# Autodesk Inventor assembly: WagonHandleAssembly
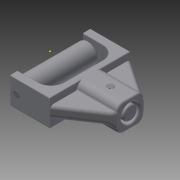
[picture p0: Inventor's stored thumbnail of the model, 180x180]
Saved by Autodesk Inventor 2014 (Build 180170000, 170)
## iProperties
Created: 2013-11-29
Part Number: WagonHandleAssembly
Document SubType Name: Assembly
Designer: steele
Author: steele
## Documents named in this file (5)
- C:\Users\steele\Google Drive\FMHS-CAD\Steele Robot Parts\WagonHandleAssembly.iam
- C:\Users\steele\Google Drive\FMHS-CAD\Steele Robot Parts\WagonHandleV02.ipt
- C:\Users\steele\Google Drive\FMHS-CAD\Steele Robot Parts\WagonHandleAssembly\Design Accelerator\Bolted Connection1.iam
- C:\Users\steele\Google Drive\FMHS-CAD\Steele Robot Parts\Wagon Hand Handle V02.ipt
- C:\Users\steele\Google Drive\FMHS-CAD\Steele Robot Parts\WagonHandleAssembly\Design Accelerator\Bolted Connection2.iam
## Components (4 placed, 4 different names)
1. WagonHandleV02:1 — Mate:1, Mate:2, Mate:3, Mate:4
2. Bolted Connection For Handle [sub-assembly] — Mate:1, Mate:2, Insert:1
3. Wagon Hand Handle V02:1 — Insert:1
4. Bolted Connection For Pipe [sub-assembly] — Mate:3, Mate:4
## Relationships (5: Mate 4, Insert 1)
- Mate:1: WagonHandleV02:1 ↔ Bolted Connection For Handle
- Mate:2: WagonHandleV02:1 ↔ Bolted Connection For Handle
- Insert:1 (-18.415 mm): Bolted Connection For Handle ↔ Wagon Hand Handle V02:1
- Mate:3: WagonHandleV02:1 ↔ Bolted Connection For Pipe
- Mate:4: WagonHandleV02:1 ↔ Bolted Connection For Pipe
